# Autodesk Inventor assembly: Pulley and Claw
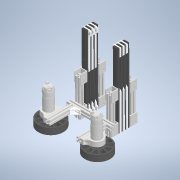
[picture p0: Inventor's stored thumbnail of the model, 180x180]
Saved by Autodesk Inventor 2020 (Build 240168000, 168)
## iProperties
Created: 2020-02-12
Part Number: Pulley and Claw
Document SubType Name: Assembly
Designer: maple
Author: maple
## Documents named in this file (5)
- C:\Users\maple\Documents\GitHub\CAD\Robotics 2019-2020\Assembly\Pulley and Claw\Pulley and Claw.iam
- C:\Users\maple\Documents\GitHub\CAD\Robotics 2019-2020\Assembly\Pulley and Claw\PulleySystem\x4_Pulley.iam
- C:\Users\maple\Documents\GitHub\CAD\Robotics 2019-2020\Assembly\Pulley and Claw\Claw\ClawAssembly.iam
- C:\Users\maple\Documents\GitHub\CAD\Robotics 2019-2020\Assembly\Pulley and Claw\PulleySystem\1inchExtrusion.ipt
- C:\Users\maple\Documents\GitHub\CAD\Robotics 2019-2020\Assembly\Pulley and Claw\PulleySystem\Long Robotics Mount V2.ipt
## Components (15 placed, 4 different names)
1. x4_Pulley:1 [sub-assembly] — Rotational:1, Rotational:2, Rotational:5, Rotational:6, Flush:3, Flush:4, Flush:7, Flush:8, Flush:9, Flush:10, Flush:11, Flush:12
2. x4_Pulley:2 [sub-assembly] — Rotational:3, Rotational:4, Rotational:7, Rotational:8, Flush:1, Flush:2, Flush:5, Flush:6, Flush:13, Flush:14, Flush:15, Flush:16
3. ClawAssembly:1 [sub-assembly] — Mate:5, Mate:6, Mate:7, Flush:17, Flush:18, Flush:21, Flush:22
4. 1inchExtrusion:1 — Mate:2, Flush:3, Flush:4, Mate:5, Flush:17, Flush:22
5. 1inchExtrusion:2 — Mate:4, Flush:7, Flush:8
6. 1inchExtrusion:3 — Mate:3, Flush:5, Flush:6
7. 1inchExtrusion:4 — Mate:1, Flush:1, Flush:2, Mate:6, Mate:7, Flush:18, Flush:21
8. Long Robotics Mount V2:1 — Rotational:3, Mate:3, Flush:15
9. Long Robotics Mount V2:2 — Rotational:4, Flush:16
10. Long Robotics Mount V2:3 — Rotational:8, Flush:13
11. Long Robotics Mount V2:4 — Rotational:7, Mate:1, Flush:14
12. Long Robotics Mount V2:5 — Rotational:2, Mate:4, Flush:9
13. Long Robotics Mount V2:6 — Rotational:6, Flush:12
14. Long Robotics Mount V2:7 — Rotational:5, Mate:2, Flush:11
15. Long Robotics Mount V2:8 — Rotational:1, Flush:10
## Relationships (35: Flush 20, RevoluteJoint 8, Mate 7)
- Rotational:1 [RevoluteJoint]: x4_Pulley:1 ↔ Long Robotics Mount V2:8
- Rotational:2 [RevoluteJoint]: x4_Pulley:1 ↔ Long Robotics Mount V2:5
- Rotational:3 [RevoluteJoint]: x4_Pulley:2 ↔ Long Robotics Mount V2:1
- Rotational:4 [RevoluteJoint]: x4_Pulley:2 ↔ Long Robotics Mount V2:2
- Rotational:5 [RevoluteJoint]: x4_Pulley:1 ↔ Long Robotics Mount V2:7
- Rotational:6 [RevoluteJoint]: x4_Pulley:1 ↔ Long Robotics Mount V2:6
- Rotational:7 [RevoluteJoint]: x4_Pulley:2 ↔ Long Robotics Mount V2:4
- Rotational:8 [RevoluteJoint]: x4_Pulley:2 ↔ Long Robotics Mount V2:3
- Mate:1 (5.08 mm): 1inchExtrusion:4 ↔ Long Robotics Mount V2:4
- Flush:1: x4_Pulley:2 ↔ 1inchExtrusion:4
- Flush:2: x4_Pulley:2 ↔ 1inchExtrusion:4
- Mate:2 (5.08 mm): 1inchExtrusion:1 ↔ Long Robotics Mount V2:7
- Flush:3: x4_Pulley:1 ↔ 1inchExtrusion:1
- Flush:4: x4_Pulley:1 ↔ 1inchExtrusion:1
- Mate:3 (5.08 mm): 1inchExtrusion:3 ↔ Long Robotics Mount V2:1
- Flush:5: x4_Pulley:2 ↔ 1inchExtrusion:3
- Flush:6: x4_Pulley:2 ↔ 1inchExtrusion:3
- Mate:4 (5.08 mm): 1inchExtrusion:2 ↔ Long Robotics Mount V2:5
- Flush:7: x4_Pulley:1 ↔ 1inchExtrusion:2
- Flush:8: x4_Pulley:1 ↔ 1inchExtrusion:2
- Flush:9 (-4.3434 mm): x4_Pulley:1 ↔ Long Robotics Mount V2:5
- Flush:10 (-4.3434 mm): x4_Pulley:1 ↔ Long Robotics Mount V2:8
- Flush:11 (-4.7244 mm): x4_Pulley:1 ↔ Long Robotics Mount V2:7
- Flush:12 (-4.7244 mm): x4_Pulley:1 ↔ Long Robotics Mount V2:6
- Flush:13 (-4.7244 mm): x4_Pulley:2 ↔ Long Robotics Mount V2:3
- Flush:14 (-4.7244 mm): x4_Pulley:2 ↔ Long Robotics Mount V2:4
- Flush:15 (-3.9624 mm): x4_Pulley:2 ↔ Long Robotics Mount V2:1
- Flush:16 (-4.3434 mm): x4_Pulley:2 ↔ Long Robotics Mount V2:2
- Mate:5: ClawAssembly:1 ↔ 1inchExtrusion:1
- Mate:6: ClawAssembly:1 ↔ 1inchExtrusion:4
- Mate:7: ClawAssembly:1 ↔ 1inchExtrusion:4
- Flush:17: ClawAssembly:1 ↔ 1inchExtrusion:1
- Flush:18: ClawAssembly:1 ↔ 1inchExtrusion:4
- Flush:21: ClawAssembly:1 ↔ 1inchExtrusion:4
- Flush:22: ClawAssembly:1 ↔ 1inchExtrusion:1
